# Autodesk Inventor assembly: HbHand
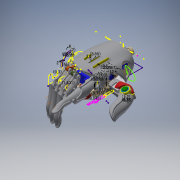
[picture p0: Inventor's stored thumbnail of the model, 180x180]
Saved by Autodesk Inventor 2018.1 (Build 221171000, 171)
## iProperties
Part Number: HbHand
Material: 一般
Document SubType Name: Assembly
Designer: sktom
Author: sktom
## Documents named in this file (37)
- D:\CloudStrage\OneDrive\CAD\MAJ\hackberry\HACKberry-hardware\3D_69%inlength\Inventor\HbHandForChild\HbHand.iam
- D:\CloudStrage\OneDrive\CAD\MAJ\hackberry\HACKberry-hardware\3D_69%inlength\Inventor\HbHandForChild\HbPalmBase03ForChild.ipt
- D:\CloudStrage\OneDrive\CAD\MAJ\hackberry\HACKberry-hardware\3D_69%inlength\Inventor\HbHandForChild\bearing_683.ipt
- D:\CloudStrage\OneDrive\CAD\MAJ\hackberry\HACKberry-hardware\3D_69%inlength\Inventor\HbHandForChild\HbthumbU02ForChild\HbthumbU02ForChild.iam
- D:\CloudStrage\OneDrive\CAD\MAJ\hackberry\HACKberry-hardware\3D_69%inlength\Inventor\HbHandForChild\HbServoHK282A\Servo_HK282A_Hone.ipt
- D:\CloudStrage\OneDrive\CAD\MAJ\hackberry\HACKberry-hardware\3D_69%inlength\Inventor\HbHandForChild\HbIndexFinger01ForChild\HbIndexFinger01ForChild.iam
- D:\CloudStrage\OneDrive\CAD\MAJ\hackberry\HACKberry-hardware\3D_69%inlength\Inventor\HbHandForChild\HbFinger01ForChild\HbFinger01ForChild.iam
- D:\CloudStrage\OneDrive\CAD\MAJ\hackberry\HACKberry-hardware\3D_69%inlength\Inventor\HbHandForChild\HbRing-LittleCouplerLink01ForChild.ipt
- D:\CloudStrage\OneDrive\CAD\MAJ\hackberry\HACKberry-hardware\3D_69%inlength\Inventor\HbHandForChild\HbMiddle-RingCouplerLink01ForChild.ipt
- D:\CloudStrage\OneDrive\CAD\MAJ\hackberry\HACKberry-hardware\3D_69%inlength\Inventor\HbHandForChild\servo\Tower Pro 9g Micro Servo SG90.iam
- D:\CloudStrage\OneDrive\CAD\MAJ\hackberry\HACKberry-hardware\3D_69%inlength\Inventor\HbHandForChild\DummyASV-15MG.ipt
- D:\CloudStrage\OneDrive\CAD\MAJ\hackberry\HACKberry-hardware\3D_69%inlength\Inventor\HbHandForChild\HbFingerMainCouplerLink01ForChild.ipt
- D:\CloudStrage\OneDrive\CAD\MAJ\hackberry\HACKberry-hardware\3D_69%inlength\Inventor\HbHandForChild\DummyASV-15MGSingleHorn01.ipt
- D:\CloudStrage\OneDrive\CAD\MAJ\hackberry\HACKberry-hardware\3D_69%inlength\Inventor\HbHandForChild\HbBackCover02ForChild.ipt
- D:\CloudStrage\OneDrive\CAD\MAJ\hackberry\HACKberry-hardware\3D_69%inlength\Inventor\HbHandForChild\Spur Gear (16 teeth).ipt
- D:\CloudStrage\OneDrive\CAD\MAJ\hackberry\HACKberry-hardware\3D_69%inlength\Inventor\HbHandForChild\spacer_2_3_l3.5.ipt
- D:\CloudStrage\OneDrive\CAD\MAJ\hackberry\HACKberry-hardware\3D_69%inlength\Inventor\HbHandForChild\HbServoCover.ipt
- D:\CloudStrage\OneDrive\CAD\MAJ\hackberry\HACKberry-hardware\3D_69%inlength\Inventor\HbHandForChild\HbShaftStopperB04ForChild.ipt
- D:\CloudStrage\OneDrive\CAD\MAJ\hackberry\HACKberry-hardware\3D_69%inlength\Inventor\HbHandForChild\HbShaftStopperA04ForChild.ipt
- D:\CloudStrage\OneDrive\CAD\MAJ\hackberry\HACKberry-hardware\3D_69%inlength\Inventor\HbHandForChild\shaft_phi1.5_l10.ipt
- D:\CloudStrage\OneDrive\CAD\MAJ\hackberry\HACKberry-hardware\3D_69%inlength\Inventor\HbHandForChild\bolt_M2L6.ipt
- D:\CloudStrage\OneDrive\CAD\MAJ\hackberry\HACKberry-hardware\3D_69%inlength\Inventor\HbHandForChild\HbCircuit\HbBoard.ipt
- D:\CloudStrage\OneDrive\CAD\MAJ\hackberry\HACKberry-hardware\3D_69%inlength\Inventor\HbHandForChild\HbPowerLever05ForChild.ipt
- D:\CloudStrage\OneDrive\CAD\MAJ\hackberry\HACKberry-hardware\3D_69%inlength\Inventor\HbHandForChild\HbSwitch\HbFingerLockButton05.ipt
- D:\CloudStrage\OneDrive\CAD\MAJ\hackberry\HACKberry-hardware\3D_69%inlength\Inventor\HbHandForChild\HbSwitch\HbMaxButton05.ipt
- D:\CloudStrage\OneDrive\CAD\MAJ\hackberry\HACKberry-hardware\3D_69%inlength\Inventor\HbHandForChild\HbSwitch\HbMinButton05.ipt
- D:\CloudStrage\OneDrive\CAD\MAJ\hackberry\HACKberry-hardware\3D_69%inlength\Inventor\HbHandForChild\HbSwitch\HbThumbButton05.ipt
- D:\CloudStrage\OneDrive\CAD\MAJ\hackberry\HACKberry-hardware\3D_69%inlength\Inventor\HbHandForChild\HbCircuit\SKRPACE010.ipt
- D:\CloudStrage\OneDrive\CAD\MAJ\hackberry\HACKberry-hardware\3D_69%inlength\Inventor\HbHandForChild\HbCircuit\IS-1250.ipt
- D:\CloudStrage\OneDrive\CAD\MAJ\hackberry\HACKberry-hardware\3D_69%inlength\Inventor\HbHandForChild\HbCircuit\530470310.ipt
- D:\CloudStrage\OneDrive\CAD\MAJ\hackberry\HACKberry-hardware\3D_69%inlength\Inventor\HbHandForChild\HbCircuit\510210300.ipt
- D:\CloudStrage\OneDrive\CAD\MAJ\hackberry\HACKberry-hardware\3D_69%inlength\Inventor\HbHandForChild\HbCircuit\Pololu_A_Star_32U4_Micro.ipt
- D:\CloudStrage\OneDrive\CAD\MAJ\hackberry\HACKberry-hardware\3D_69%inlength\Inventor\HbHandForChild\HbCircuit\S2B-PH-K-S.ipt
- D:\CloudStrage\OneDrive\CAD\MAJ\hackberry\HACKberry-hardware\3D_69%inlength\Inventor\HbHandForChild\HbCircuit\PHR-2.ipt
- D:\CloudStrage\OneDrive\CAD\MAJ\hackberry\HACKberry-hardware\3D_69%inlength\Inventor\HbHandForChild\HbCircuit\S3B-PH-K-S.ipt
- D:\CloudStrage\OneDrive\CAD\MAJ\hackberry\HACKberry-hardware\3D_69%inlength\Inventor\HbHandForChild\bolt_M1.4L6.ipt
- D:\CloudStrage\OneDrive\CAD\MAJ\hackberry\HACKberry-hardware\3D_69%inlength\Inventor\HbHandForChild\S7V7F5.ipt
## Components (62 placed, 36 different names)
1. HbPalmBase03ForChild:1 — 挿入:1, 挿入:4, 挿入:5, 挿入:6, 挿入:7, 挿入:8, 挿入:9, 挿入:10, 挿入:11, 挿入:12, 挿入:15, 挿入:16, メイト:2, メイト:3, 挿入:22, 挿入:23, 挿入:31, 挿入:32, 挿入:33, 挿入:34, 挿入:35, 挿入:36, 挿入:37, 挿入:38, 挿入:39, 挿入:40, 挿入:41, フラッシュ:3, メイト:26, メイト:32, メイト:33, メイト:34, メイト:35
2. bearing_683:1 — 挿入:1, 挿入:2
3. HbthumbU02ForChild:1 [sub-assembly] — 挿入:2, 挿入:3
4. Servo_HK282A_Hone:1 — 挿入:3, 挿入:4, 挿入:5, 挿入:52, 挿入:53
5. HbIndexFinger01ForChild:1 [sub-assembly] — 挿入:6
6. HbFinger01ForChild:1 [sub-assembly] — 挿入:7, 挿入:8, 挿入:30
7. HbFinger01ForChild:2 [sub-assembly] — 挿入:9, 挿入:10, 挿入:28, 挿入:29
8. HbFinger01ForChild:3 [sub-assembly] — 挿入:11, 挿入:12, 挿入:19, 挿入:26, 挿入:27
9. HbRing-LittleCouplerLink01ForChild:1 — 円柱状:5, 円柱状:6, フラッシュ:2, 挿入:46, 挿入:47
10. HbMiddle-RingCouplerLink01ForChild:1 — 円柱状:3, 円柱状:4, フラッシュ:1
11. Tower Pro 9g Micro Servo SG90:1 [sub-assembly] — 挿入:15, 挿入:16, 挿入:24
12. DummyASV-15MG:1 — 挿入:20, メイト:2, メイト:3
13. HbFingerMainCouplerLink01ForChild:1 — 挿入:19, 挿入:42, 挿入:43
14. DummyASV-15MGSingleHorn01:1 — 挿入:20, 挿入:42
15. HbBackCover02ForChild:1 — 挿入:22, 挿入:23, メイト:4, メイト:5, メイト:6, メイト:7, メイト:10, メイト:11
16. Spur Gear (16 teeth):1 — 挿入:24
17. spacer_2_3_l3.5:1 — 挿入:26
18. spacer_2_3_l3.5:2 — 挿入:43, 挿入:48
19. spacer_2_3_l3.5:3 — 挿入:27, 円柱状:6, フラッシュ:2
20. spacer_2_3_l3.5:4 — 挿入:28, 円柱状:5
21. spacer_2_3_l3.5:5 — 挿入:29, 円柱状:3, フラッシュ:1, 挿入:45
22. spacer_2_3_l3.5:6 — 挿入:30, 円柱状:4, 挿入:44
23. HbServoCover:1 — 挿入:31, 挿入:32, 挿入:49, 挿入:50, 挿入:51
24. HbShaftStopperB04ForChild:1 — 挿入:34
25. HbShaftStopperA04ForChild:1 — 挿入:33
26. shaft_phi1.5_l10:1 — 挿入:35
27. shaft_phi1.5_l10:2 — 挿入:36
28. shaft_phi1.5_l10:3 — 挿入:37
29. shaft_phi1.5_l10:4 — 挿入:38
30. shaft_phi1.5_l10:5 — 挿入:39
31. shaft_phi1.5_l10:6 — 挿入:41
32. shaft_phi1.5_l10:7 — 挿入:40
33. bolt_M2L6:1 — 挿入:44
34. bolt_M2L6:2 — 挿入:45
35. bolt_M2L6:3 — 挿入:46
36. bolt_M2L6:4 — 挿入:47
37. bolt_M2L6:5 — 挿入:48
38. HbBoard:1 — フラッシュ:3, メイト:12, メイト:13, メイト:14, メイト:15, メイト:16, メイト:20, フラッシュ:13, メイト:21, メイト:22, メイト:25, フラッシュ:18, フラッシュ:19, メイト:29, フラッシュ:20, メイト:30
39. HbPowerLever05ForChild:1 — メイト:4, メイト:5
40. HbFingerLockButton05:1 — メイト:6, メイト:7
41. HbMaxButton05:1 — フラッシュ:6, フラッシュ:7, メイト:8
42. HbMinButton05:1 — フラッシュ:4, フラッシュ:5, フラッシュ:6, フラッシュ:7, メイト:8, メイト:9, メイト:10, メイト:11
43. HbThumbButton05:1 — フラッシュ:4, フラッシュ:5, メイト:9
44. SKRPACE010:1 — メイト:12, フラッシュ:8, フラッシュ:10, フラッシュ:12
45. SKRPACE010:2 — メイト:14, フラッシュ:8, フラッシュ:9, フラッシュ:10, フラッシュ:11
46. SKRPACE010:3 — メイト:13, フラッシュ:12
47. SKRPACE010:4 — メイト:15, フラッシュ:9, フラッシュ:11
48. IS-1250:1 — メイト:16
49. 530470310:1 — メイト:17, メイト:18, メイト:19, メイト:20, フラッシュ:13, フラッシュ:14, フラッシュ:15, メイト:23
50. 510210300:1 — メイト:17, メイト:18, メイト:19
51. 530470310:2 — フラッシュ:14, メイト:21, メイト:23, メイト:24
52. 530470310:3 — フラッシュ:15, メイト:22, メイト:24
53. bolt_M1.4L6:3 — 挿入:51
54. bolt_M1.4L6:2 — 挿入:50
55. bolt_M1.4L6:1 — 挿入:49
56. S2B-PH-K-S:1 — メイト:25, フラッシュ:18, メイト:26, メイト:27, メイト:28
57. PHR-2:1 — メイト:27, メイト:28
58. Pololu_A_Star_32U4_Micro:1 — フラッシュ:19, メイト:29, フラッシュ:20
59. S3B-PH-K-S:1 — メイト:30, メイト:32
60. bolt_M1.4L6:4 — 挿入:53
61. bolt_M1.4L6:5 — 挿入:52
62. S7V7F5:1 — メイト:33, メイト:34, メイト:35
## Relationships (102: Insert 47, Mate 33, Flush 18, CylindricalJoint 4)
- 挿入:1 [Insert]: HbPalmBase03ForChild:1 ↔ bearing_683:1
- 挿入:2 [Insert]: bearing_683:1 ↔ HbthumbU02ForChild:1
- 挿入:3 [Insert]: HbthumbU02ForChild:1 ↔ Servo_HK282A_Hone:1
- 挿入:4 [Insert]: HbPalmBase03ForChild:1 ↔ Servo_HK282A_Hone:1
- 挿入:5 [Insert]: HbPalmBase03ForChild:1 ↔ Servo_HK282A_Hone:1
- 挿入:6 [Insert]: HbPalmBase03ForChild:1 ↔ HbIndexFinger01ForChild:1
- 挿入:7 [Insert]: HbPalmBase03ForChild:1 ↔ HbFinger01ForChild:1
- 挿入:8 [Insert]: HbPalmBase03ForChild:1 ↔ HbFinger01ForChild:1
- 挿入:9 [Insert]: HbPalmBase03ForChild:1 ↔ HbFinger01ForChild:2
- 挿入:10 [Insert]: HbPalmBase03ForChild:1 ↔ HbFinger01ForChild:2
- 挿入:11 [Insert]: HbPalmBase03ForChild:1 ↔ HbFinger01ForChild:3
- 挿入:12 [Insert]: HbPalmBase03ForChild:1 ↔ HbFinger01ForChild:3
- 挿入:15 [Insert]: HbPalmBase03ForChild:1 ↔ Tower Pro 9g Micro Servo SG90:1
- 挿入:16 [Insert]: HbPalmBase03ForChild:1 ↔ Tower Pro 9g Micro Servo SG90:1
- 挿入:19 [Insert] (0.1 mm): HbFinger01ForChild:3 ↔ HbFingerMainCouplerLink01ForChild:1
- 挿入:20 [Insert]: DummyASV-15MG:1 ↔ DummyASV-15MGSingleHorn01:1
- メイト:2 [Mate]: HbPalmBase03ForChild:1 ↔ DummyASV-15MG:1
- メイト:3 [Mate]: HbPalmBase03ForChild:1 ↔ DummyASV-15MG:1
- 挿入:22 [Insert]: HbPalmBase03ForChild:1 ↔ HbBackCover02ForChild:1
- 挿入:23 [Insert]: HbPalmBase03ForChild:1 ↔ HbBackCover02ForChild:1
- 挿入:24 [Insert]: Tower Pro 9g Micro Servo SG90:1 ↔ Spur Gear (16 teeth):1
- 挿入:26 [Insert]: HbFinger01ForChild:3 ↔ spacer_2_3_l3.5:1
- 挿入:27 [Insert]: HbFinger01ForChild:3 ↔ spacer_2_3_l3.5:3
- 挿入:28 [Insert]: HbFinger01ForChild:2 ↔ spacer_2_3_l3.5:4
- 挿入:29 [Insert]: HbFinger01ForChild:2 ↔ spacer_2_3_l3.5:5
- 挿入:30 [Insert]: HbFinger01ForChild:1 ↔ spacer_2_3_l3.5:6
- 挿入:31 [Insert]: HbPalmBase03ForChild:1 ↔ HbServoCover:1
- 挿入:32 [Insert]: HbPalmBase03ForChild:1 ↔ HbServoCover:1
- 挿入:33 [Insert]: HbPalmBase03ForChild:1 ↔ HbShaftStopperA04ForChild:1
- 挿入:34 [Insert]: HbPalmBase03ForChild:1 ↔ HbShaftStopperB04ForChild:1
- 挿入:35 [Insert]: HbPalmBase03ForChild:1 ↔ shaft_phi1.5_l10:1
- 挿入:36 [Insert] (0.5 mm): HbPalmBase03ForChild:1 ↔ shaft_phi1.5_l10:2
- 挿入:37 [Insert] (0.3 mm): HbPalmBase03ForChild:1 ↔ shaft_phi1.5_l10:3
- 挿入:38 [Insert] (0.3 mm): HbPalmBase03ForChild:1 ↔ shaft_phi1.5_l10:4
- 挿入:39 [Insert] (0.5 mm): HbPalmBase03ForChild:1 ↔ shaft_phi1.5_l10:5
- 挿入:40 [Insert] (0.5 mm): HbPalmBase03ForChild:1 ↔ shaft_phi1.5_l10:7
- 挿入:41 [Insert] (0.5 mm): HbPalmBase03ForChild:1 ↔ shaft_phi1.5_l10:6
- 挿入:42 [Insert]: HbFingerMainCouplerLink01ForChild:1 ↔ DummyASV-15MGSingleHorn01:1
- 挿入:43 [Insert]: HbFingerMainCouplerLink01ForChild:1 ↔ spacer_2_3_l3.5:2
- 円柱状:3 [CylindricalJoint]: HbMiddle-RingCouplerLink01ForChild:1 ↔ spacer_2_3_l3.5:5
- 円柱状:4 [CylindricalJoint]: HbMiddle-RingCouplerLink01ForChild:1 ↔ spacer_2_3_l3.5:6
- 挿入:44 [Insert] (0.3 mm): spacer_2_3_l3.5:6 ↔ bolt_M2L6:1
- フラッシュ:1 [Flush]: HbMiddle-RingCouplerLink01ForChild:1 ↔ spacer_2_3_l3.5:5
- 挿入:45 [Insert] (0.3 mm): spacer_2_3_l3.5:5 ↔ bolt_M2L6:2
- 円柱状:5 [CylindricalJoint]: HbRing-LittleCouplerLink01ForChild:1 ↔ spacer_2_3_l3.5:4
- 円柱状:6 [CylindricalJoint]: HbRing-LittleCouplerLink01ForChild:1 ↔ spacer_2_3_l3.5:3
- フラッシュ:2 [Flush]: HbRing-LittleCouplerLink01ForChild:1 ↔ spacer_2_3_l3.5:3
- 挿入:46 [Insert] (0.3 mm): HbRing-LittleCouplerLink01ForChild:1 ↔ bolt_M2L6:3
- 挿入:47 [Insert] (0.3 mm): HbRing-LittleCouplerLink01ForChild:1 ↔ bolt_M2L6:4
- 挿入:48 [Insert] (0.3 mm): spacer_2_3_l3.5:2 ↔ bolt_M2L6:5
- フラッシュ:3 [Flush]: HbPalmBase03ForChild:1 ↔ HbBoard:1
- メイト:4 [Mate] (0.3 mm): HbBackCover02ForChild:1 ↔ HbPowerLever05ForChild:1
- メイト:5 [Mate] (0.5 mm): HbBackCover02ForChild:1 ↔ HbPowerLever05ForChild:1
- メイト:6 [Mate] (0.5 mm): HbBackCover02ForChild:1 ↔ HbFingerLockButton05:1
- メイト:7 [Mate] (0.25 mm): HbBackCover02ForChild:1 ↔ HbFingerLockButton05:1
- フラッシュ:4 [Flush]: HbMinButton05:1 ↔ HbThumbButton05:1
- フラッシュ:5 [Flush]: HbMinButton05:1 ↔ HbThumbButton05:1
- フラッシュ:6 [Flush]: HbMaxButton05:1 ↔ HbMinButton05:1
- フラッシュ:7 [Flush]: HbMaxButton05:1 ↔ HbMinButton05:1
- メイト:8 [Mate] (0.25 mm): HbMaxButton05:1 ↔ HbMinButton05:1
- メイト:9 [Mate] (0.25 mm): HbMinButton05:1 ↔ HbThumbButton05:1
- メイト:10 [Mate] (0.5 mm): HbBackCover02ForChild:1 ↔ HbMinButton05:1
- メイト:11 [Mate] (0.25 mm): HbBackCover02ForChild:1 ↔ HbMinButton05:1
- メイト:12 [Mate]: HbBoard:1 ↔ SKRPACE010:1
- メイト:13 [Mate]: HbBoard:1 ↔ SKRPACE010:3
- メイト:14 [Mate]: HbBoard:1 ↔ SKRPACE010:2
- メイト:15 [Mate]: HbBoard:1 ↔ SKRPACE010:4
- フラッシュ:8 [Flush]: SKRPACE010:1 ↔ SKRPACE010:2
- フラッシュ:9 [Flush]: SKRPACE010:2 ↔ SKRPACE010:4
- フラッシュ:10 [Flush] (-7.8 mm): SKRPACE010:1 ↔ SKRPACE010:2
- フラッシュ:11 [Flush] (-7.8 mm): SKRPACE010:2 ↔ SKRPACE010:4
- フラッシュ:12 [Flush] (17.911 mm): SKRPACE010:1 ↔ SKRPACE010:3
- メイト:16 [Mate]: HbBoard:1 ↔ IS-1250:1
- メイト:17 [Mate]: 530470310:1 ↔ 510210300:1
- メイト:18 [Mate]: 530470310:1 ↔ 510210300:1
- メイト:19 [Mate] (0.4 mm): 530470310:1 ↔ 510210300:1
- メイト:20 [Mate]: HbBoard:1 ↔ 530470310:1
- フラッシュ:13 [Flush] (-0.5 mm): HbBoard:1 ↔ 530470310:1
- フラッシュ:14 [Flush]: 530470310:1 ↔ 530470310:2
- フラッシュ:15 [Flush]: 530470310:1 ↔ 530470310:3
- メイト:21 [Mate]: HbBoard:1 ↔ 530470310:2
- メイト:22 [Mate]: HbBoard:1 ↔ 530470310:3
- メイト:23 [Mate] (0.8 mm): 530470310:1 ↔ 530470310:2
- メイト:24 [Mate] (0.8 mm): 530470310:2 ↔ 530470310:3
- 挿入:49 [Insert]: HbServoCover:1 ↔ bolt_M1.4L6:1
- 挿入:50 [Insert]: HbServoCover:1 ↔ bolt_M1.4L6:2
- 挿入:51 [Insert]: HbServoCover:1 ↔ bolt_M1.4L6:3
- メイト:25 [Mate]: HbBoard:1 ↔ S2B-PH-K-S:1
- フラッシュ:18 [Flush] (2 mm): HbBoard:1 ↔ S2B-PH-K-S:1
- メイト:26 [Mate] (0.5 mm): HbPalmBase03ForChild:1 ↔ S2B-PH-K-S:1
- メイト:27 [Mate]: S2B-PH-K-S:1 ↔ PHR-2:1
- メイト:28 [Mate]: S2B-PH-K-S:1 ↔ PHR-2:1
- フラッシュ:19 [Flush] (-3 mm): HbBoard:1 ↔ Pololu_A_Star_32U4_Micro:1
- メイト:29 [Mate] (2 mm): HbBoard:1 ↔ Pololu_A_Star_32U4_Micro:1
- フラッシュ:20 [Flush]: HbBoard:1 ↔ Pololu_A_Star_32U4_Micro:1
- メイト:30 [Mate]: HbBoard:1 ↔ S3B-PH-K-S:1
- 挿入:52 [Insert]: Servo_HK282A_Hone:1 ↔ bolt_M1.4L6:5
- 挿入:53 [Insert]: Servo_HK282A_Hone:1 ↔ bolt_M1.4L6:4
- メイト:32 [Mate] (-2 mm): HbPalmBase03ForChild:1 ↔ S3B-PH-K-S:1
- メイト:33 [Mate]: HbPalmBase03ForChild:1 ↔ S7V7F5:1
- メイト:34 [Mate]: HbPalmBase03ForChild:1 ↔ S7V7F5:1
- メイト:35 [Mate]: HbPalmBase03ForChild:1 ↔ S7V7F5:1
